# Autodesk Inventor assembly: 6in traction wheel assy
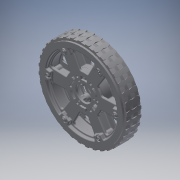
[picture p0: Inventor's stored thumbnail of the model, 180x180]
Saved by Autodesk Inventor 2016 (Build 200138000, 138)
## iProperties
Created: 2013-12-10
Part Number: 6in traction wheel assy
Description: STEP AP214
Document SubType Name: Assembly
Designer: blake
Sending System: SolidWorks 2013
Preprocessor: SwSTEP 2.0
Title: 217-2860-STEP.STEP
Revision Number: ANY
## Documents named in this file (3)
- C:\Users\blake\Documents\24 hour CAD\engineering library\hardware\wheels\6in traction wheel assy.iam
- C:\Users\blake\Documents\24 hour CAD\engineering library\hardware\wheels\217-2860-001 Rev3.ipt
- C:\Users\blake\Documents\24 hour CAD\engineering library\hardware\wheels\6in traction wheel.iam
## Components (3 placed, 3 different names)
1. 217-2860-001 Rev3_1 — Mate:2, Mate:4
2. 6in traction wheel:1 [sub-assembly] — Mate:2, Mate:3, Mate:4, Mate:5
3. 217-2860-001 Rev3:2 — Mate:3, Mate:5
## Relationships (4: Mate 4)
- Mate:2: 217-2860-001 Rev3_1 ↔ 6in traction wheel:1
- Mate:3: 6in traction wheel:1 ↔ 217-2860-001 Rev3:2
- Mate:4: 217-2860-001 Rev3_1 ↔ 6in traction wheel:1
- Mate:5: 6in traction wheel:1 ↔ 217-2860-001 Rev3:2
